# Autodesk Inventor assembly: sumobotLIDAR
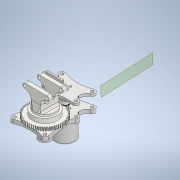
[picture p0: Inventor's stored thumbnail of the model, 180x180]
Saved by Autodesk Inventor 2022 (Build 260153070, 153G)
## iProperties
Created: 2021-10-27
Part Number: sumobotLIDAR
Document SubType Name: Assembly
Designer: a laptop
Mass: 24.9045 g
Surface Area: 154.1 cm^2
Volume: 24.9045 cm^3
Density: 1 g/cm^3
Author: a laptop
## Documents named in this file (11)
- C:\Users\a laptop\Desktop\SumoBot\sumobotLIDAR\sumobotLIDAR.iam
- C:\Users\a laptop\Desktop\SumoBot\sumobotLIDAR\MOTOR.ipt
- C:\Users\a laptop\Desktop\SumoBot\sumobotLIDAR\SRM-12-06A.ipt
- C:\Users\a laptop\Desktop\SumoBot\sumobotLIDAR\Adapterlowerplate.ipt
- C:\Users\a laptop\Desktop\SumoBot\sumobotLIDAR\608ZZ bearing.ipt
- C:\Users\a laptop\Desktop\SumoBot\sumobotLIDAR\VL53L1X board.ipt
- C:\Users\a laptop\Desktop\SumoBot\sumobotLIDAR\AS5600.ipt
- C:\Users\a laptop\Desktop\SumoBot\sumobotLIDAR\Magnet.ipt
- C:\Users\a laptop\Desktop\SumoBot\sumobotLIDAR\MotorGear.ipt
- C:\Users\a laptop\Desktop\SumoBot\sumobotLIDAR\sumobotLIDAR\Design Accelerator\Spur Gears3.iam
- C:\Users\a laptop\Desktop\SumoBot\sumobotLIDAR\AS5600_mount.ipt
## Components (10 placed, 10 different names)
1. MOTOR:1 — Angle:1, Flush:1, Mate:5, Mate:6, Mate:7, Tangent:1, Flush:3, Mate:18, Mate:32, Flush:8, Mate:49
2. SRM-12-06A:1 — Angle:1, Flush:1, Mate:1, Mate:2, Mate:10, Mate:13, Tangent:1, Mate:14, Mate:17
3. Adapterlowerplate:1 — Flush:3, Mate:16, Mate:17, Mate:18, Mate:39, Mate:40, Mate:41, Mate:42, Flush:14
4. 608ZZ bearing:1 — Mate:15, Mate:16, Mate:48
5. VL53L1X board:1 — Mate:55, Mate:56, Mate:57
6. AS5600:1 — Mate:25, Mate:26, Mate:27, Mate:28, Angle:4, Flush:7, Mate:38, Flush:13, Mate:50, Mate:51
7. Magnet:1 — Flush:7, Flush:11
8. MotorGear:1 — Flush:8
9. Spur Gears:1 [sub-assembly] — Flush:14, Flush:11, Flush:12, Mate:48, Mate:49, Mate:55, Mate:56, Mate:57
10. AS5600_mount:1 — Flush:13, Mate:50, Mate:51
## Relationships (59: Mate 44, Flush 9, Angle 4, Tangent 1, Symmetry 1)
- Angle:1 (180 deg): MOTOR:1 ↔ SRM-12-06A:1
- Flush:1: MOTOR:1 ↔ SRM-12-06A:1
- Mate:1: SRM-12-06A:1
- Mate:2: SRM-12-06A:1
- Mate:3
- Mate:4
- Mate:5: MOTOR:1
- Mate:6: MOTOR:1
- Mate:7: MOTOR:1
- Mate:8
- Mate:9
- Flush:2 (17 mm)
- Angle:2 (180 deg)
- Mate:10: SRM-12-06A:1
- Mate:11
- Mate:12
- Angle:3 (90 deg)
- Mate:13: SRM-12-06A:1
- Tangent:1: MOTOR:1 ↔ SRM-12-06A:1
- Flush:3: MOTOR:1 ↔ Adapterlowerplate:1
- Mate:14: SRM-12-06A:1
- Mate:15: 608ZZ bearing:1
- Mate:16: Adapterlowerplate:1 ↔ 608ZZ bearing:1
- Mate:17: SRM-12-06A:1 ↔ Adapterlowerplate:1
- Mate:18: MOTOR:1 ↔ Adapterlowerplate:1
- Mate:25: AS5600:1
- Mate:26: AS5600:1
- Mate:27: AS5600:1
- Mate:28: AS5600:1
- Mate:29
- Mate:30
- Mate:31
- Angle:4 (0 deg): AS5600:1
- Mate:32: MOTOR:1
- Flush:7 (1.5 mm): AS5600:1 ↔ Magnet:1
- Flush:8: MOTOR:1 ↔ MotorGear:1
- Flush:14 (-1 mm): Adapterlowerplate:1 ↔ Spur Gears:1
- Flush:11: Magnet:1 ↔ Spur Gears:1
- Flush:12: Spur Gears:1
- Mate:38: AS5600:1
- Mate:39: Adapterlowerplate:1
- Mate:40: Adapterlowerplate:1
- Mate:41: Adapterlowerplate:1
- Mate:42: Adapterlowerplate:1
- Mate:43
- Mate:44
- Mate:45
- Mate:46
- Symmetry:1
- Mate:47
- Flush:13: AS5600:1 ↔ AS5600_mount:1
- Mate:48: 608ZZ bearing:1 ↔ Spur Gears:1
- Mate:49: MOTOR:1 ↔ Spur Gears:1
- Mate:50: AS5600:1 ↔ AS5600_mount:1
- Mate:51: AS5600:1 ↔ AS5600_mount:1
- Mate:54
- Mate:55: VL53L1X board:1 ↔ Spur Gears:1
- Mate:56: VL53L1X board:1 ↔ Spur Gears:1
- Mate:57: VL53L1X board:1 ↔ Spur Gears:1
